# Autodesk Inventor assembly: 08-20-2023 assieme ganascia con blocco
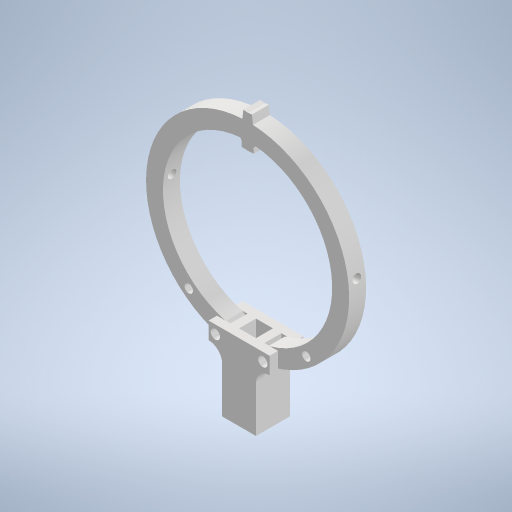
[picture p0: Inventor's stored thumbnail of the model, 512x512]
Saved by Autodesk Inventor 2023 (Build 270158000, 158)
## iProperties
Created: 2023-08-20
Part Number: 08-20-2023 assieme ganascia con blocco
Document SubType Name: Assembly
Designer: Admin
Author: Admin
## Documents named in this file (3)
- C:\Users\Admin\Desktop\3DDDD\da stampanre\08-01-2023 pezzi per pinza telescopica\08-20-2023 assieme ganascia con blocco.iam
- C:\Users\Admin\Desktop\3DDDD\da stampanre\08-01-2023 pezzi per pinza telescopica\asta con serraggio pinza.ipt
- C:\Users\Admin\Desktop\3DDDD\da stampanre\08-01-2023 pezzi per pinza telescopica\ganascia.ipt
## Components (3 placed, 2 different names)
1. asta con serraggio pinza:1 — Coincidente:1, Coincidente:2, Coincidente:3, Coincidente:4
2. ganascia:1 — Coincidente:3, Coincidente:4
3. ganascia:2 — Coincidente:1, Coincidente:2
## Relationships (4: Mate 4)
- Coincidente:1 [Mate]: asta con serraggio pinza:1 ↔ ganascia:2
- Coincidente:2 [Mate]: asta con serraggio pinza:1 ↔ ganascia:2
- Coincidente:3 [Mate]: asta con serraggio pinza:1 ↔ ganascia:1
- Coincidente:4 [Mate]: asta con serraggio pinza:1 ↔ ganascia:1
